# Autodesk Inventor assembly: PLANCHAS PARA CORTAR
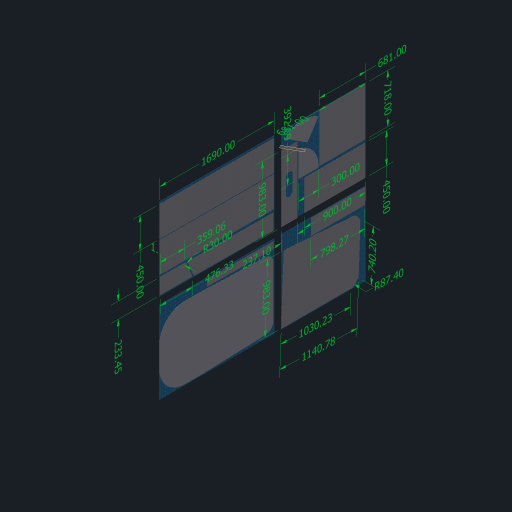
[picture p0: Inventor's stored thumbnail of the model, 512x512]
Saved by Autodesk Inventor 2024.3 (Build 283343000, 343)
## iProperties
Created: 2024-05-15
Part Number: PLANCHAS PARA CORTAR
Material: Generic
Document SubType Name: Assembly
Designer: Niler
Author: Niler
## Documents named in this file (15)
- C:\Users\Niler\OneDrive\Escritorio\RECICLADOR\RECICLADOR_MODELO_3D\VERSION_3_COMPLETA\NUEVAS_CHAPAS_ALUMINIO\PLANCHAS PARA CORTAR_NUEVO.iam
- C:\Users\Niler\OneDrive\Escritorio\RECICLADOR\RECICLADOR_MODELO_3D\VERSION_3_COMPLETA\NUEVAS_CHAPAS_ALUMINIO\PLANCHA_1-7.ipt
- C:\Users\Niler\OneDrive\Escritorio\RECICLADOR\RECICLADOR_MODELO_3D\VERSION_3_COMPLETA\NUEVAS_CHAPAS_ALUMINIO\PLANCHA_1-3.ipt
- C:\Users\Niler\OneDrive\Escritorio\RECICLADOR\RECICLADOR_MODELO_3D\VERSION_3_COMPLETA\NUEVAS_CHAPAS_ALUMINIO\CHAPA_2.ipt
- C:\Users\Niler\OneDrive\Escritorio\RECICLADOR\RECICLADOR_MODELO_3D\VERSION_3_COMPLETA\NUEVAS_CHAPAS_ALUMINIO\CHAPA_3.ipt
- C:\Users\Niler\OneDrive\Escritorio\RECICLADOR\RECICLADOR_MODELO_3D\VERSION_3_COMPLETA\NUEVAS_CHAPAS_ALUMINIO\CHAPA_6.ipt
- C:\Users\Niler\OneDrive\Escritorio\RECICLADOR\RECICLADOR_MODELO_3D\VERSION_3_COMPLETA\NUEVAS_CHAPAS_ALUMINIO\CHAPA_5.ipt
- C:\Users\Niler\OneDrive\Escritorio\RECICLADOR\RECICLADOR_MODELO_3D\VERSION_3_COMPLETA\NUEVAS_CHAPAS_ALUMINIO\CHAPA_7.ipt
- C:\Users\Niler\OneDrive\Escritorio\RECICLADOR\RECICLADOR_MODELO_3D\VERSION_3_COMPLETA\NUEVAS_CHAPAS_ALUMINIO\AUX_LARGO.ipt
- C:\Users\Niler\OneDrive\Escritorio\RECICLADOR\RECICLADOR_MODELO_3D\VERSION_3_COMPLETA\NUEVAS_CHAPAS_ALUMINIO\AUX_LARGO_P2.ipt
- C:\Users\Niler\OneDrive\Escritorio\RECICLADOR\RECICLADOR_MODELO_3D\VERSION_3_COMPLETA\NUEVAS_CHAPAS_ALUMINIO\AUX_2.ipt
- C:\Users\Niler\OneDrive\Escritorio\RECICLADOR\RECICLADOR_MODELO_3D\VERSION_3_COMPLETA\NUEVAS_CHAPAS_ALUMINIO\AUX_2._MIRipt.ipt
- C:\Users\Niler\OneDrive\Escritorio\RECICLADOR\RECICLADOR_MODELO_3D\VERSION_3_COMPLETA\NUEVAS_CHAPAS_ALUMINIO\AUX_3.ipt
- C:\Users\Niler\OneDrive\Escritorio\RECICLADOR\RECICLADOR_MODELO_3D\VERSION_3_COMPLETA\NUEVAS_CHAPAS_ALUMINIO\AUX_4.ipt
- C:\Users\Niler\OneDrive\Escritorio\RECICLADOR\RECICLADOR_MODELO_3D\VERSION_3_COMPLETA\NUEVAS_CHAPAS_ALUMINIO\AUX_2 _P2.ipt
## Components (18 placed, 14 different names)
1. PLANCHA_1-7:1 — Flush:1, Mate:1, Flush:4, Flush:5, Mate:3, Flush:6, Mate:7, Flush:8
2. PLANCHA_1-7:2 — Flush:5, Mate:3, Flush:6
3. PLANCHA_1-3:1 — Flush:1, Flush:2, Flush:3, Mate:1, Mate:2, Flush:4, Mate:8, Mate:10, Mate:11
4. PLANCHA_1-3:2 — Flush:2, Flush:3, Mate:2, Mate:6, Mate:12
5. CHAPA_2:1 — Mate:5
6. CHAPA_3:1 — Mate:5, Mate:6
7. CHAPA_6:1 — Mate:7, Flush:8
8. CHAPA_5:1 — Mate:8
9. CHAPA_7:1 — Mate:10
10. AUX_LARGO:1
11. AUX_LARGO_P2:1 — Mate:11
12. AUX_LARGO:2
13. AUX_2:1
14. AUX_2._MIRipt:1
15. AUX_3:1
16. CHAPA_7:2 — Mate:12
17. AUX_4:1
18. AUX_2 _P2:1
## Relationships (19: Mate 11, Flush 8)
- Flush:1: PLANCHA_1-7:1 ↔ PLANCHA_1-3:1
- Flush:2: PLANCHA_1-3:1 ↔ PLANCHA_1-3:2
- Flush:3: PLANCHA_1-3:1 ↔ PLANCHA_1-3:2
- Mate:1 (100 mm): PLANCHA_1-7:1 ↔ PLANCHA_1-3:1
- Mate:2 (100 mm): PLANCHA_1-3:1 ↔ PLANCHA_1-3:2
- Flush:4: PLANCHA_1-7:1 ↔ PLANCHA_1-3:1
- Flush:5: PLANCHA_1-7:1 ↔ PLANCHA_1-7:2
- Mate:3 (100 mm): PLANCHA_1-7:1 ↔ PLANCHA_1-7:2
- Flush:6: PLANCHA_1-7:1 ↔ PLANCHA_1-7:2
- [Mate]: CHAPA_2:1 ↔ CHAPA_3:1
- [Flush]: CHAPA_2:1 ↔ CHAPA_3:1
- Mate:5: CHAPA_2:1 ↔ CHAPA_3:1
- Mate:6: PLANCHA_1-3:2 ↔ CHAPA_3:1
- Mate:7: PLANCHA_1-7:1 ↔ CHAPA_6:1
- Flush:8: PLANCHA_1-7:1 ↔ CHAPA_6:1
- Mate:8: PLANCHA_1-3:1 ↔ CHAPA_5:1
- Mate:10: PLANCHA_1-3:1 ↔ CHAPA_7:1
- Mate:11: PLANCHA_1-3:1 ↔ AUX_LARGO_P2:1
- Mate:12: PLANCHA_1-3:2 ↔ CHAPA_7:2
